# Autodesk Inventor assembly: FRC Fixed Field 2018_sldasm
(part 2 of 4)
- C:\Users\CAD\Documents\GitHub\FIRST-ROBOTICS-2018-5436-CAD\Field\FIRST Power Up Field CAD\Body_858_sldprt.ipt
- C:\Users\CAD\Documents\GitHub\FIRST-ROBOTICS-2018-5436-CAD\Field\FIRST Power Up Field CAD\Body_859_sldprt.ipt
- C:\Users\CAD\Documents\GitHub\FIRST-ROBOTICS-2018-5436-CAD\Field\FIRST Power Up Field CAD\Body_860_sldprt.ipt
- C:\Users\CAD\Documents\GitHub\FIRST-ROBOTICS-2018-5436-CAD\Field\FIRST Power Up Field CAD\Body_861_sldprt.ipt
- C:\Users\CAD\Documents\GitHub\FIRST-ROBOTICS-2018-5436-CAD\Field\FIRST Power Up Field CAD\Body_862_sldprt.ipt
- C:\Users\CAD\Documents\GitHub\FIRST-ROBOTICS-2018-5436-CAD\Field\FIRST Power Up Field CAD\Body_863_sldprt.ipt
- C:\Users\CAD\Documents\GitHub\FIRST-ROBOTICS-2018-5436-CAD\Field\FIRST Power Up Field CAD\Body_864_sldprt.ipt
- C:\Users\CAD\Documents\GitHub\FIRST-ROBOTICS-2018-5436-CAD\Field\FIRST Power Up Field CAD\Body_865_sldprt.ipt
- C:\Users\CAD\Documents\GitHub\FIRST-ROBOTICS-2018-5436-CAD\Field\FIRST Power Up Field CAD\Body_866_sldprt.ipt
- C:\Users\CAD\Documents\GitHub\FIRST-ROBOTICS-2018-5436-CAD\Field\FIRST Power Up Field CAD\Body_867_sldprt.ipt
- C:\Users\CAD\Documents\GitHub\FIRST-ROBOTICS-2018-5436-CAD\Field\FIRST Power Up Field CAD\Body_868_sldprt.ipt
- C:\Users\CAD\Documents\GitHub\FIRST-ROBOTICS-2018-5436-CAD\Field\FIRST Power Up Field CAD\Body_869_sldprt.ipt
- C:\Users\CAD\Documents\GitHub\FIRST-ROBOTICS-2018-5436-CAD\Field\FIRST Power Up Field CAD\Body_870_sldprt.ipt
- C:\Users\CAD\Documents\GitHub\FIRST-ROBOTICS-2018-5436-CAD\Field\FIRST Power Up Field CAD\Body_871_sldprt.ipt
- C:\Users\CAD\Documents\GitHub\FIRST-ROBOTICS-2018-5436-CAD\Field\FIRST Power Up Field CAD\Body_872_sldprt.ipt
- C:\Users\CAD\Documents\GitHub\FIRST-ROBOTICS-2018-5436-CAD\Field\FIRST Power Up Field CAD\Body_873_sldprt.ipt
- C:\Users\CAD\Documents\GitHub\FIRST-ROBOTICS-2018-5436-CAD\Field\FIRST Power Up Field CAD\Body_874_sldprt.ipt
- C:\Users\CAD\Documents\GitHub\FIRST-ROBOTICS-2018-5436-CAD\Field\FIRST Power Up Field CAD\Body_875_sldprt.ipt
- C:\Users\CAD\Documents\GitHub\FIRST-ROBOTICS-2018-5436-CAD\Field\FIRST Power Up Field CAD\Body_876_sldprt.ipt
- C:\Users\CAD\Documents\GitHub\FIRST-ROBOTICS-2018-5436-CAD\Field\FIRST Power Up Field CAD\Body_877_sldprt.ipt
- C:\Users\CAD\Documents\GitHub\FIRST-ROBOTICS-2018-5436-CAD\Field\FIRST Power Up Field CAD\Body_878_sldprt.ipt
- C:\Users\CAD\Documents\GitHub\FIRST-ROBOTICS-2018-5436-CAD\Field\FIRST Power Up Field CAD\Body_879_sldprt.ipt
- C:\Users\CAD\Documents\GitHub\FIRST-ROBOTICS-2018-5436-CAD\Field\FIRST Power Up Field CAD\Body_880_sldprt.ipt
- C:\Users\CAD\Documents\GitHub\FIRST-ROBOTICS-2018-5436-CAD\Field\FIRST Power Up Field CAD\Body_881_sldprt.ipt
- C:\Users\CAD\Documents\GitHub\FIRST-ROBOTICS-2018-5436-CAD\Field\FIRST Power Up Field CAD\Body_882_sldprt.ipt
- C:\Users\CAD\Documents\GitHub\FIRST-ROBOTICS-2018-5436-CAD\Field\FIRST Power Up Field CAD\Body_883_sldprt.ipt
- C:\Users\CAD\Documents\GitHub\FIRST-ROBOTICS-2018-5436-CAD\Field\FIRST Power Up Field CAD\Body_884_sldprt.ipt
- C:\Users\CAD\Documents\GitHub\FIRST-ROBOTICS-2018-5436-CAD\Field\FIRST Power Up Field CAD\Body_885_sldprt.ipt
- C:\Users\CAD\Documents\GitHub\FIRST-ROBOTICS-2018-5436-CAD\Field\FIRST Power Up Field CAD\Body_886_sldprt.ipt
- C:\Users\CAD\Documents\GitHub\FIRST-ROBOTICS-2018-5436-CAD\Field\FIRST Power Up Field CAD\Body_887_sldprt.ipt
- C:\Users\CAD\Documents\GitHub\FIRST-ROBOTICS-2018-5436-CAD\Field\FIRST Power Up Field CAD\Body_888_sldprt.ipt
- C:\Users\CAD\Documents\GitHub\FIRST-ROBOTICS-2018-5436-CAD\Field\FIRST Power Up Field CAD\Body_889_sldprt.ipt
- C:\Users\CAD\Documents\GitHub\FIRST-ROBOTICS-2018-5436-CAD\Field\FIRST Power Up Field CAD\Body_890_sldprt.ipt
- C:\Users\CAD\Documents\GitHub\FIRST-ROBOTICS-2018-5436-CAD\Field\FIRST Power Up Field CAD\Body_891_sldprt.ipt
- C:\Users\CAD\Documents\GitHub\FIRST-ROBOTICS-2018-5436-CAD\Field\FIRST Power Up Field CAD\Body_892_sldprt.ipt
- C:\Users\CAD\Documents\GitHub\FIRST-ROBOTICS-2018-5436-CAD\Field\FIRST Power Up Field CAD\Body_893_sldprt.ipt
- C:\Users\CAD\Documents\GitHub\FIRST-ROBOTICS-2018-5436-CAD\Field\FIRST Power Up Field CAD\Body_894_sldprt.ipt
- C:\Users\CAD\Documents\GitHub\FIRST-ROBOTICS-2018-5436-CAD\Field\FIRST Power Up Field CAD\Body_895_sldprt.ipt
- C:\Users\CAD\Documents\GitHub\FIRST-ROBOTICS-2018-5436-CAD\Field\FIRST Power Up Field CAD\Body_896_sldprt.ipt
- C:\Users\CAD\Documents\GitHub\FIRST-ROBOTICS-2018-5436-CAD\Field\FIRST Power Up Field CAD\Body_897_sldprt.ipt
- C:\Users\CAD\Documents\GitHub\FIRST-ROBOTICS-2018-5436-CAD\Field\FIRST Power Up Field CAD\Body_898_sldprt.ipt
- C:\Users\CAD\Documents\GitHub\FIRST-ROBOTICS-2018-5436-CAD\Field\FIRST Power Up Field CAD\Body_899_sldprt.ipt
- C:\Users\CAD\Documents\GitHub\FIRST-ROBOTICS-2018-5436-CAD\Field\FIRST Power Up Field CAD\Body_900_sldprt.ipt
- C:\Users\CAD\Documents\GitHub\FIRST-ROBOTICS-2018-5436-CAD\Field\FIRST Power Up Field CAD\Body_901_sldprt.ipt
- C:\Users\CAD\Documents\GitHub\FIRST-ROBOTICS-2018-5436-CAD\Field\FIRST Power Up Field CAD\Body_902_sldprt.ipt
- C:\Users\CAD\Documents\GitHub\FIRST-ROBOTICS-2018-5436-CAD\Field\FIRST Power Up Field CAD\Body_903_sldprt.ipt
- C:\Users\CAD\Documents\GitHub\FIRST-ROBOTICS-2018-5436-CAD\Field\FIRST Power Up Field CAD\Body_904_sldprt.ipt
- C:\Users\CAD\Documents\GitHub\FIRST-ROBOTICS-2018-5436-CAD\Field\FIRST Power Up Field CAD\Body_905_sldprt.ipt
- C:\Users\CAD\Documents\GitHub\FIRST-ROBOTICS-2018-5436-CAD\Field\FIRST Power Up Field CAD\Body_906_sldprt.ipt
- C:\Users\CAD\Documents\GitHub\FIRST-ROBOTICS-2018-5436-CAD\Field\FIRST Power Up Field CAD\Body_907_sldprt.ipt
- C:\Users\CAD\Documents\GitHub\FIRST-ROBOTICS-2018-5436-CAD\Field\FIRST Power Up Field CAD\Body_908_sldprt.ipt
- C:\Users\CAD\Documents\GitHub\FIRST-ROBOTICS-2018-5436-CAD\Field\FIRST Power Up Field CAD\Body_909_sldprt.ipt
- C:\Users\CAD\Documents\GitHub\FIRST-ROBOTICS-2018-5436-CAD\Field\FIRST Power Up Field CAD\Body_910_sldprt.ipt
- C:\Users\CAD\Documents\GitHub\FIRST-ROBOTICS-2018-5436-CAD\Field\FIRST Power Up Field CAD\Body_911_sldprt.ipt
- C:\Users\CAD\Documents\GitHub\FIRST-ROBOTICS-2018-5436-CAD\Field\FIRST Power Up Field CAD\Body_912_sldprt.ipt
- C:\Users\CAD\Documents\GitHub\FIRST-ROBOTICS-2018-5436-CAD\Field\FIRST Power Up Field CAD\Body_913_sldprt.ipt
- C:\Users\CAD\Documents\GitHub\FIRST-ROBOTICS-2018-5436-CAD\Field\FIRST Power Up Field CAD\Body_914_sldprt.ipt
- C:\Users\CAD\Documents\GitHub\FIRST-ROBOTICS-2018-5436-CAD\Field\FIRST Power Up Field CAD\Body_915_sldprt.ipt
- C:\Users\CAD\Documents\GitHub\FIRST-ROBOTICS-2018-5436-CAD\Field\FIRST Power Up Field CAD\Body_916_sldprt.ipt
- C:\Users\CAD\Documents\GitHub\FIRST-ROBOTICS-2018-5436-CAD\Field\FIRST Power Up Field CAD\Body_917_sldprt.ipt
- C:\Users\CAD\Documents\GitHub\FIRST-ROBOTICS-2018-5436-CAD\Field\FIRST Power Up Field CAD\Body_918_sldprt.ipt
- C:\Users\CAD\Documents\GitHub\FIRST-ROBOTICS-2018-5436-CAD\Field\FIRST Power Up Field CAD\Body_919_sldprt.ipt
- C:\Users\CAD\Documents\GitHub\FIRST-ROBOTICS-2018-5436-CAD\Field\FIRST Power Up Field CAD\Body_920_sldprt.ipt
- C:\Users\CAD\Documents\GitHub\FIRST-ROBOTICS-2018-5436-CAD\Field\FIRST Power Up Field CAD\Body_921_sldprt.ipt
- C:\Users\CAD\Documents\GitHub\FIRST-ROBOTICS-2018-5436-CAD\Field\FIRST Power Up Field CAD\Body_922_sldprt.ipt
- C:\Users\CAD\Documents\GitHub\FIRST-ROBOTICS-2018-5436-CAD\Field\FIRST Power Up Field CAD\Body_923_sldprt.ipt
- C:\Users\CAD\Documents\GitHub\FIRST-ROBOTICS-2018-5436-CAD\Field\FIRST Power Up Field CAD\Body_924_sldprt.ipt
- C:\Users\CAD\Documents\GitHub\FIRST-ROBOTICS-2018-5436-CAD\Field\FIRST Power Up Field CAD\Body_925_sldprt.ipt
- C:\Users\CAD\Documents\GitHub\FIRST-ROBOTICS-2018-5436-CAD\Field\FIRST Power Up Field CAD\Body_926_sldprt.ipt
- C:\Users\CAD\Documents\GitHub\FIRST-ROBOTICS-2018-5436-CAD\Field\FIRST Power Up Field CAD\Body_927_sldprt.ipt
- C:\Users\CAD\Documents\GitHub\FIRST-ROBOTICS-2018-5436-CAD\Field\FIRST Power Up Field CAD\Body_928_sldprt.ipt
- C:\Users\CAD\Documents\GitHub\FIRST-ROBOTICS-2018-5436-CAD\Field\FIRST Power Up Field CAD\Body_929_sldprt.ipt
- C:\Users\CAD\Documents\GitHub\FIRST-ROBOTICS-2018-5436-CAD\Field\FIRST Power Up Field CAD\Body_930_sldprt.ipt
- C:\Users\CAD\Documents\GitHub\FIRST-ROBOTICS-2018-5436-CAD\Field\FIRST Power Up Field CAD\Body_931_sldprt.ipt
- C:\Users\CAD\Documents\GitHub\FIRST-ROBOTICS-2018-5436-CAD\Field\FIRST Power Up Field CAD\Body_932_sldprt.ipt
- C:\Users\CAD\Documents\GitHub\FIRST-ROBOTICS-2018-5436-CAD\Field\FIRST Power Up Field CAD\Body_933_sldprt.ipt
- C:\Users\CAD\Documents\GitHub\FIRST-ROBOTICS-2018-5436-CAD\Field\FIRST Power Up Field CAD\Body_934_sldprt.ipt
- C:\Users\CAD\Documents\GitHub\FIRST-ROBOTICS-2018-5436-CAD\Field\FIRST Power Up Field CAD\Body_935_sldprt.ipt
- C:\Users\CAD\Documents\GitHub\FIRST-ROBOTICS-2018-5436-CAD\Field\FIRST Power Up Field CAD\Body_936_sldprt.ipt
- C:\Users\CAD\Documents\GitHub\FIRST-ROBOTICS-2018-5436-CAD\Field\FIRST Power Up Field CAD\Body_937_sldprt.ipt
- C:\Users\CAD\Documents\GitHub\FIRST-ROBOTICS-2018-5436-CAD\Field\FIRST Power Up Field CAD\Body_938_sldprt.ipt
- C:\Users\CAD\Documents\GitHub\FIRST-ROBOTICS-2018-5436-CAD\Field\FIRST Power Up Field CAD\Body_939_sldprt.ipt
- C:\Users\CAD\Documents\GitHub\FIRST-ROBOTICS-2018-5436-CAD\Field\FIRST Power Up Field CAD\Body_940_sldprt.ipt
- C:\Users\CAD\Documents\GitHub\FIRST-ROBOTICS-2018-5436-CAD\Field\FIRST Power Up Field CAD\Body_941_sldprt.ipt
- C:\Users\CAD\Documents\GitHub\FIRST-ROBOTICS-2018-5436-CAD\Field\FIRST Power Up Field CAD\Body_942_sldprt.ipt
- C:\Users\CAD\Documents\GitHub\FIRST-ROBOTICS-2018-5436-CAD\Field\FIRST Power Up Field CAD\Body_943_sldprt.ipt
- C:\Users\CAD\Documents\GitHub\FIRST-ROBOTICS-2018-5436-CAD\Field\FIRST Power Up Field CAD\Body_944_sldprt.ipt
- C:\Users\CAD\Documents\GitHub\FIRST-ROBOTICS-2018-5436-CAD\Field\FIRST Power Up Field CAD\Body_945_sldprt.ipt
- C:\Users\CAD\Documents\GitHub\FIRST-ROBOTICS-2018-5436-CAD\Field\FIRST Power Up Field CAD\Body_946_sldprt.ipt
- C:\Users\CAD\Documents\GitHub\FIRST-ROBOTICS-2018-5436-CAD\Field\FIRST Power Up Field CAD\Body_947_sldprt.ipt
- C:\Users\CAD\Documents\GitHub\FIRST-ROBOTICS-2018-5436-CAD\Field\FIRST Power Up Field CAD\Body_948_sldprt.ipt
- C:\Users\CAD\Documents\GitHub\FIRST-ROBOTICS-2018-5436-CAD\Field\FIRST Power Up Field CAD\Body_949_sldprt.ipt
- C:\Users\CAD\Documents\GitHub\FIRST-ROBOTICS-2018-5436-CAD\Field\FIRST Power Up Field CAD\Body_950_sldprt.ipt
- C:\Users\CAD\Documents\GitHub\FIRST-ROBOTICS-2018-5436-CAD\Field\FIRST Power Up Field CAD\Body_951_sldprt.ipt
- C:\Users\CAD\Documents\GitHub\FIRST-ROBOTICS-2018-5436-CAD\Field\FIRST Power Up Field CAD\Body_952_sldprt.ipt
- C:\Users\CAD\Documents\GitHub\FIRST-ROBOTICS-2018-5436-CAD\Field\FIRST Power Up Field CAD\Body_953_sldprt.ipt
- C:\Users\CAD\Documents\GitHub\FIRST-ROBOTICS-2018-5436-CAD\Field\FIRST Power Up Field CAD\Body_954_sldprt.ipt
- C:\Users\CAD\Documents\GitHub\FIRST-ROBOTICS-2018-5436-CAD\Field\FIRST Power Up Field CAD\Body_955_sldprt.ipt
- C:\Users\CAD\Documents\GitHub\FIRST-ROBOTICS-2018-5436-CAD\Field\FIRST Power Up Field CAD\Body_956_sldprt.ipt
- C:\Users\CAD\Documents\GitHub\FIRST-ROBOTICS-2018-5436-CAD\Field\FIRST Power Up Field CAD\Body_957_sldprt.ipt
- C:\Users\CAD\Documents\GitHub\FIRST-ROBOTICS-2018-5436-CAD\Field\FIRST Power Up Field CAD\Body_958_sldprt.ipt
- C:\Users\CAD\Documents\GitHub\FIRST-ROBOTICS-2018-5436-CAD\Field\FIRST Power Up Field CAD\Body_959_sldprt.ipt
- C:\Users\CAD\Documents\GitHub\FIRST-ROBOTICS-2018-5436-CAD\Field\FIRST Power Up Field CAD\Body_960_sldprt.ipt
- C:\Users\CAD\Documents\GitHub\FIRST-ROBOTICS-2018-5436-CAD\Field\FIRST Power Up Field CAD\Body_961_sldprt.ipt
- C:\Users\CAD\Documents\GitHub\FIRST-ROBOTICS-2018-5436-CAD\Field\FIRST Power Up Field CAD\Body_962_sldprt.ipt
- C:\Users\CAD\Documents\GitHub\FIRST-ROBOTICS-2018-5436-CAD\Field\FIRST Power Up Field CAD\Body_963_sldprt.ipt
- C:\Users\CAD\Documents\GitHub\FIRST-ROBOTICS-2018-5436-CAD\Field\FIRST Power Up Field CAD\Body_964_sldprt.ipt
- C:\Users\CAD\Documents\GitHub\FIRST-ROBOTICS-2018-5436-CAD\Field\FIRST Power Up Field CAD\Body_965_sldprt.ipt
- C:\Users\CAD\Documents\GitHub\FIRST-ROBOTICS-2018-5436-CAD\Field\FIRST Power Up Field CAD\Body_966_sldprt.ipt
- C:\Users\CAD\Documents\GitHub\FIRST-ROBOTICS-2018-5436-CAD\Field\FIRST Power Up Field CAD\Body_967_sldprt.ipt
- C:\Users\CAD\Documents\GitHub\FIRST-ROBOTICS-2018-5436-CAD\Field\FIRST Power Up Field CAD\Body_968_sldprt.ipt
- C:\Users\CAD\Documents\GitHub\FIRST-ROBOTICS-2018-5436-CAD\Field\FIRST Power Up Field CAD\Body_969_sldprt.ipt
- C:\Users\CAD\Documents\GitHub\FIRST-ROBOTICS-2018-5436-CAD\Field\FIRST Power Up Field CAD\Body_970_sldprt.ipt
- C:\Users\CAD\Documents\GitHub\FIRST-ROBOTICS-2018-5436-CAD\Field\FIRST Power Up Field CAD\Body_971_sldprt.ipt
- C:\Users\CAD\Documents\GitHub\FIRST-ROBOTICS-2018-5436-CAD\Field\FIRST Power Up Field CAD\Body_972_sldprt.ipt
- C:\Users\CAD\Documents\GitHub\FIRST-ROBOTICS-2018-5436-CAD\Field\FIRST Power Up Field CAD\Body_973_sldprt.ipt
- C:\Users\CAD\Documents\GitHub\FIRST-ROBOTICS-2018-5436-CAD\Field\FIRST Power Up Field CAD\Body_974_sldprt.ipt
- C:\Users\CAD\Documents\GitHub\FIRST-ROBOTICS-2018-5436-CAD\Field\FIRST Power Up Field CAD\Body_975_sldprt.ipt
- C:\Users\CAD\Documents\GitHub\FIRST-ROBOTICS-2018-5436-CAD\Field\FIRST Power Up Field CAD\Body_976_sldprt.ipt
- C:\Users\CAD\Documents\GitHub\FIRST-ROBOTICS-2018-5436-CAD\Field\FIRST Power Up Field CAD\Body_977_sldprt.ipt
- C:\Users\CAD\Documents\GitHub\FIRST-ROBOTICS-2018-5436-CAD\Field\FIRST Power Up Field CAD\Body_978_sldprt.ipt
- C:\Users\CAD\Documents\GitHub\FIRST-ROBOTICS-2018-5436-CAD\Field\FIRST Power Up Field CAD\Body_979_sldprt.ipt
- C:\Users\CAD\Documents\GitHub\FIRST-ROBOTICS-2018-5436-CAD\Field\FIRST Power Up Field CAD\Body_980_sldprt.ipt
- C:\Users\CAD\Documents\GitHub\FIRST-ROBOTICS-2018-5436-CAD\Field\FIRST Power Up Field CAD\Body_981_sldprt.ipt
- C:\Users\CAD\Documents\GitHub\FIRST-ROBOTICS-2018-5436-CAD\Field\FIRST Power Up Field CAD\Body_982_sldprt.ipt
- C:\Users\CAD\Documents\GitHub\FIRST-ROBOTICS-2018-5436-CAD\Field\FIRST Power Up Field CAD\Body_983_sldprt.ipt
- C:\Users\CAD\Documents\GitHub\FIRST-ROBOTICS-2018-5436-CAD\Field\FIRST Power Up Field CAD\Body_984_sldprt.ipt
- C:\Users\CAD\Documents\GitHub\FIRST-ROBOTICS-2018-5436-CAD\Field\FIRST Power Up Field CAD\Body_985_sldprt.ipt
- C:\Users\CAD\Documents\GitHub\FIRST-ROBOTICS-2018-5436-CAD\Field\FIRST Power Up Field CAD\Body_986_sldprt.ipt
- C:\Users\CAD\Documents\GitHub\FIRST-ROBOTICS-2018-5436-CAD\Field\FIRST Power Up Field CAD\Body_987_sldprt.ipt
- C:\Users\CAD\Documents\GitHub\FIRST-ROBOTICS-2018-5436-CAD\Field\FIRST Power Up Field CAD\Body_988_sldprt.ipt
- C:\Users\CAD\Documents\GitHub\FIRST-ROBOTICS-2018-5436-CAD\Field\FIRST Power Up Field CAD\Body_989_sldprt.ipt
- C:\Users\CAD\Documents\GitHub\FIRST-ROBOTICS-2018-5436-CAD\Field\FIRST Power Up Field CAD\Body_990_sldprt.ipt
- C:\Users\CAD\Documents\GitHub\FIRST-ROBOTICS-2018-5436-CAD\Field\FIRST Power Up Field CAD\Body_991_sldprt.ipt
- C:\Users\CAD\Documents\GitHub\FIRST-ROBOTICS-2018-5436-CAD\Field\FIRST Power Up Field CAD\Body_992_sldprt.ipt
- C:\Users\CAD\Documents\GitHub\FIRST-ROBOTICS-2018-5436-CAD\Field\FIRST Power Up Field CAD\Body_993_sldprt.ipt
- C:\Users\CAD\Documents\GitHub\FIRST-ROBOTICS-2018-5436-CAD\Field\FIRST Power Up Field CAD\Body_994_sldprt.ipt
- C:\Users\CAD\Documents\GitHub\FIRST-ROBOTICS-2018-5436-CAD\Field\FIRST Power Up Field CAD\Body_995_sldprt.ipt
- C:\Users\CAD\Documents\GitHub\FIRST-ROBOTICS-2018-5436-CAD\Field\FIRST Power Up Field CAD\Body_996_sldprt.ipt
- C:\Users\CAD\Documents\GitHub\FIRST-ROBOTICS-2018-5436-CAD\Field\FIRST Power Up Field CAD\Body_997_sldprt.ipt
- C:\Users\CAD\Documents\GitHub\FIRST-ROBOTICS-2018-5436-CAD\Field\FIRST Power Up Field CAD\Body_998_sldprt.ipt
- C:\Users\CAD\Documents\GitHub\FIRST-ROBOTICS-2018-5436-CAD\Field\FIRST Power Up Field CAD\Body_999_sldprt.ipt
- C:\Users\CAD\Documents\GitHub\FIRST-ROBOTICS-2018-5436-CAD\Field\FIRST Power Up Field CAD\Body_1000_sldprt.ipt
- C:\Users\CAD\Documents\GitHub\FIRST-ROBOTICS-2018-5436-CAD\Field\FIRST Power Up Field CAD\Body_1001_sldprt.ipt
- C:\Users\CAD\Documents\GitHub\FIRST-ROBOTICS-2018-5436-CAD\Field\FIRST Power Up Field CAD\Body_1002_sldprt.ipt
- C:\Users\CAD\Documents\GitHub\FIRST-ROBOTICS-2018-5436-CAD\Field\FIRST Power Up Field CAD\Body_1003_sldprt.ipt
- C:\Users\CAD\Documents\GitHub\FIRST-ROBOTICS-2018-5436-CAD\Field\FIRST Power Up Field CAD\Body_1004_sldprt.ipt
- C:\Users\CAD\Documents\GitHub\FIRST-ROBOTICS-2018-5436-CAD\Field\FIRST Power Up Field CAD\Body_1005_sldprt.ipt
- C:\Users\CAD\Documents\GitHub\FIRST-ROBOTICS-2018-5436-CAD\Field\FIRST Power Up Field CAD\Body_1006_sldprt.ipt
- C:\Users\CAD\Documents\GitHub\FIRST-ROBOTICS-2018-5436-CAD\Field\FIRST Power Up Field CAD\Body_1007_sldprt.ipt
- C:\Users\CAD\Documents\GitHub\FIRST-ROBOTICS-2018-5436-CAD\Field\FIRST Power Up Field CAD\Body_1008_sldprt.ipt
- C:\Users\CAD\Documents\GitHub\FIRST-ROBOTICS-2018-5436-CAD\Field\FIRST Power Up Field CAD\Body_1009_sldprt.ipt
- C:\Users\CAD\Documents\GitHub\FIRST-ROBOTICS-2018-5436-CAD\Field\FIRST Power Up Field CAD\Body_1010_sldprt.ipt
- C:\Users\CAD\Documents\GitHub\FIRST-ROBOTICS-2018-5436-CAD\Field\FIRST Power Up Field CAD\Body_1011_sldprt.ipt
- C:\Users\CAD\Documents\GitHub\FIRST-ROBOTICS-2018-5436-CAD\Field\FIRST Power Up Field CAD\Body_1012_sldprt.ipt
- C:\Users\CAD\Documents\GitHub\FIRST-ROBOTICS-2018-5436-CAD\Field\FIRST Power Up Field CAD\Body_1013_sldprt.ipt
- C:\Users\CAD\Documents\GitHub\FIRST-ROBOTICS-2018-5436-CAD\Field\FIRST Power Up Field CAD\Body_1014_sldprt.ipt
- C:\Users\CAD\Documents\GitHub\FIRST-ROBOTICS-2018-5436-CAD\Field\FIRST Power Up Field CAD\Body_1015_sldprt.ipt
- C:\Users\CAD\Documents\GitHub\FIRST-ROBOTICS-2018-5436-CAD\Field\FIRST Power Up Field CAD\Body_1016_sldprt.ipt
- C:\Users\CAD\Documents\GitHub\FIRST-ROBOTICS-2018-5436-CAD\Field\FIRST Power Up Field CAD\Body_1017_sldprt.ipt
- C:\Users\CAD\Documents\GitHub\FIRST-ROBOTICS-2018-5436-CAD\Field\FIRST Power Up Field CAD\Body_1018_sldprt.ipt
- C:\Users\CAD\Documents\GitHub\FIRST-ROBOTICS-2018-5436-CAD\Field\FIRST Power Up Field CAD\Body_1019_sldprt.ipt
- C:\Users\CAD\Documents\GitHub\FIRST-ROBOTICS-2018-5436-CAD\Field\FIRST Power Up Field CAD\Body_1020_sldprt.ipt
- C:\Users\CAD\Documents\GitHub\FIRST-ROBOTICS-2018-5436-CAD\Field\FIRST Power Up Field CAD\Body_1021_sldprt.ipt
- C:\Users\CAD\Documents\GitHub\FIRST-ROBOTICS-2018-5436-CAD\Field\FIRST Power Up Field CAD\Body_1022_sldprt.ipt
- C:\Users\CAD\Documents\GitHub\FIRST-ROBOTICS-2018-5436-CAD\Field\FIRST Power Up Field CAD\Body_1023_sldprt.ipt
- C:\Users\CAD\Documents\GitHub\FIRST-ROBOTICS-2018-5436-CAD\Field\FIRST Power Up Field CAD\Body_1024_sldprt.ipt
- C:\Users\CAD\Documents\GitHub\FIRST-ROBOTICS-2018-5436-CAD\Field\FIRST Power Up Field CAD\Body_1025_sldprt.ipt
- C:\Users\CAD\Documents\GitHub\FIRST-ROBOTICS-2018-5436-CAD\Field\FIRST Power Up Field CAD\Body_1026_sldprt.ipt
- C:\Users\CAD\Documents\GitHub\FIRST-ROBOTICS-2018-5436-CAD\Field\FIRST Power Up Field CAD\Body_1027_sldprt.ipt
- C:\Users\CAD\Documents\GitHub\FIRST-ROBOTICS-2018-5436-CAD\Field\FIRST Power Up Field CAD\Body_1028_sldprt.ipt
- C:\Users\CAD\Documents\GitHub\FIRST-ROBOTICS-2018-5436-CAD\Field\FIRST Power Up Field CAD\Body_1029_sldprt.ipt
- C:\Users\CAD\Documents\GitHub\FIRST-ROBOTICS-2018-5436-CAD\Field\FIRST Power Up Field CAD\Body_1030_sldprt.ipt
- C:\Users\CAD\Documents\GitHub\FIRST-ROBOTICS-2018-5436-CAD\Field\FIRST Power Up Field CAD\Body_1031_sldprt.ipt
- C:\Users\CAD\Documents\GitHub\FIRST-ROBOTICS-2018-5436-CAD\Field\FIRST Power Up Field CAD\Body_1032_sldprt.ipt
- C:\Users\CAD\Documents\GitHub\FIRST-ROBOTICS-2018-5436-CAD\Field\FIRST Power Up Field CAD\Body_1033_sldprt.ipt
- C:\Users\CAD\Documents\GitHub\FIRST-ROBOTICS-2018-5436-CAD\Field\FIRST Power Up Field CAD\Body_1034_sldprt.ipt
- C:\Users\CAD\Documents\GitHub\FIRST-ROBOTICS-2018-5436-CAD\Field\FIRST Power Up Field CAD\Body_1035_sldprt.ipt
- C:\Users\CAD\Documents\GitHub\FIRST-ROBOTICS-2018-5436-CAD\Field\FIRST Power Up Field CAD\Body_1036_sldprt.ipt
- C:\Users\CAD\Documents\GitHub\FIRST-ROBOTICS-2018-5436-CAD\Field\FIRST Power Up Field CAD\Body_1037_sldprt.ipt
- C:\Users\CAD\Documents\GitHub\FIRST-ROBOTICS-2018-5436-CAD\Field\FIRST Power Up Field CAD\Body_1038_sldprt.ipt
- C:\Users\CAD\Documents\GitHub\FIRST-ROBOTICS-2018-5436-CAD\Field\FIRST Power Up Field CAD\Body_1039_sldprt.ipt
- C:\Users\CAD\Documents\GitHub\FIRST-ROBOTICS-2018-5436-CAD\Field\FIRST Power Up Field CAD\Body_1040_sldprt.ipt
- C:\Users\CAD\Documents\GitHub\FIRST-ROBOTICS-2018-5436-CAD\Field\FIRST Power Up Field CAD\Body_1041_sldprt.ipt
- C:\Users\CAD\Documents\GitHub\FIRST-ROBOTICS-2018-5436-CAD\Field\FIRST Power Up Field CAD\Body_1042_sldprt.ipt
- C:\Users\CAD\Documents\GitHub\FIRST-ROBOTICS-2018-5436-CAD\Field\FIRST Power Up Field CAD\Body_1043_sldprt.ipt
- C:\Users\CAD\Documents\GitHub\FIRST-ROBOTICS-2018-5436-CAD\Field\FIRST Power Up Field CAD\Body_1044_sldprt.ipt
- C:\Users\CAD\Documents\GitHub\FIRST-ROBOTICS-2018-5436-CAD\Field\FIRST Power Up Field CAD\Body_1045_sldprt.ipt
- C:\Users\CAD\Documents\GitHub\FIRST-ROBOTICS-2018-5436-CAD\Field\FIRST Power Up Field CAD\Body_1046_sldprt.ipt
- C:\Users\CAD\Documents\GitHub\FIRST-ROBOTICS-2018-5436-CAD\Field\FIRST Power Up Field CAD\Body_1047_sldprt.ipt
- C:\Users\CAD\Documents\GitHub\FIRST-ROBOTICS-2018-5436-CAD\Field\FIRST Power Up Field CAD\Body_1048_sldprt.ipt
- C:\Users\CAD\Documents\GitHub\FIRST-ROBOTICS-2018-5436-CAD\Field\FIRST Power Up Field CAD\Body_1049_sldprt.ipt
- C:\Users\CAD\Documents\GitHub\FIRST-ROBOTICS-2018-5436-CAD\Field\FIRST Power Up Field CAD\Body_1050_sldprt.ipt
- C:\Users\CAD\Documents\GitHub\FIRST-ROBOTICS-2018-5436-CAD\Field\FIRST Power Up Field CAD\Body_1051_sldprt.ipt
- C:\Users\CAD\Documents\GitHub\FIRST-ROBOTICS-2018-5436-CAD\Field\FIRST Power Up Field CAD\Body_1052_sldprt.ipt
- C:\Users\CAD\Documents\GitHub\FIRST-ROBOTICS-2018-5436-CAD\Field\FIRST Power Up Field CAD\Body_1053_sldprt.ipt
- C:\Users\CAD\Documents\GitHub\FIRST-ROBOTICS-2018-5436-CAD\Field\FIRST Power Up Field CAD\Body_1054_sldprt.ipt
- C:\Users\CAD\Documents\GitHub\FIRST-ROBOTICS-2018-5436-CAD\Field\FIRST Power Up Field CAD\Body_1055_sldprt.ipt
- C:\Users\CAD\Documents\GitHub\FIRST-ROBOTICS-2018-5436-CAD\Field\FIRST Power Up Field CAD\Body_1056_sldprt.ipt
- C:\Users\CAD\Documents\GitHub\FIRST-ROBOTICS-2018-5436-CAD\Field\FIRST Power Up Field CAD\Body_1057_sldprt.ipt
- C:\Users\CAD\Documents\GitHub\FIRST-ROBOTICS-2018-5436-CAD\Field\FIRST Power Up Field CAD\Body_1058_sldprt.ipt
- C:\Users\CAD\Documents\GitHub\FIRST-ROBOTICS-2018-5436-CAD\Field\FIRST Power Up Field CAD\Body_1059_sldprt.ipt
- C:\Users\CAD\Documents\GitHub\FIRST-ROBOTICS-2018-5436-CAD\Field\FIRST Power Up Field CAD\Body_1060_sldprt.ipt
- C:\Users\CAD\Documents\GitHub\FIRST-ROBOTICS-2018-5436-CAD\Field\FIRST Power Up Field CAD\Body_1061_sldprt.ipt
- C:\Users\CAD\Documents\GitHub\FIRST-ROBOTICS-2018-5436-CAD\Field\FIRST Power Up Field CAD\Body_1062_sldprt.ipt
- C:\Users\CAD\Documents\GitHub\FIRST-ROBOTICS-2018-5436-CAD\Field\FIRST Power Up Field CAD\Body_1063_sldprt.ipt
- C:\Users\CAD\Documents\GitHub\FIRST-ROBOTICS-2018-5436-CAD\Field\FIRST Power Up Field CAD\Body_1064_sldprt.ipt
- C:\Users\CAD\Documents\GitHub\FIRST-ROBOTICS-2018-5436-CAD\Field\FIRST Power Up Field CAD\Body_1065_sldprt.ipt
- C:\Users\CAD\Documents\GitHub\FIRST-ROBOTICS-2018-5436-CAD\Field\FIRST Power Up Field CAD\Body_1066_sldprt.ipt
- C:\Users\CAD\Documents\GitHub\FIRST-ROBOTICS-2018-5436-CAD\Field\FIRST Power Up Field CAD\Body_1067_sldprt.ipt
- C:\Users\CAD\Documents\GitHub\FIRST-ROBOTICS-2018-5436-CAD\Field\FIRST Power Up Field CAD\Body_1068_sldprt.ipt
- C:\Users\CAD\Documents\GitHub\FIRST-ROBOTICS-2018-5436-CAD\Field\FIRST Power Up Field CAD\Body_1069_sldprt.ipt
- C:\Users\CAD\Documents\GitHub\FIRST-ROBOTICS-2018-5436-CAD\Field\FIRST Power Up Field CAD\Body_1070_sldprt.ipt
- C:\Users\CAD\Documents\GitHub\FIRST-ROBOTICS-2018-5436-CAD\Field\FIRST Power Up Field CAD\Body_1071_sldprt.ipt
- C:\Users\CAD\Documents\GitHub\FIRST-ROBOTICS-2018-5436-CAD\Field\FIRST Power Up Field CAD\Body_1072_sldprt.ipt
- C:\Users\CAD\Documents\GitHub\FIRST-ROBOTICS-2018-5436-CAD\Field\FIRST Power Up Field CAD\Body_1073_sldprt.ipt
- C:\Users\CAD\Documents\GitHub\FIRST-ROBOTICS-2018-5436-CAD\Field\FIRST Power Up Field CAD\Body_1074_sldprt.ipt
- C:\Users\CAD\Documents\GitHub\FIRST-ROBOTICS-2018-5436-CAD\Field\FIRST Power Up Field CAD\Body_1075_sldprt.ipt
- C:\Users\CAD\Documents\GitHub\FIRST-ROBOTICS-2018-5436-CAD\Field\FIRST Power Up Field CAD\Body_1076_sldprt.ipt
- C:\Users\CAD\Documents\GitHub\FIRST-ROBOTICS-2018-5436-CAD\Field\FIRST Power Up Field CAD\Body_1077_sldprt.ipt
- C:\Users\CAD\Documents\GitHub\FIRST-ROBOTICS-2018-5436-CAD\Field\FIRST Power Up Field CAD\Body_1078_sldprt.ipt
- C:\Users\CAD\Documents\GitHub\FIRST-ROBOTICS-2018-5436-CAD\Field\FIRST Power Up Field CAD\Body_1079_sldprt.ipt
- C:\Users\CAD\Documents\GitHub\FIRST-ROBOTICS-2018-5436-CAD\Field\FIRST Power Up Field CAD\Body_1080_sldprt.ipt
- C:\Users\CAD\Documents\GitHub\FIRST-ROBOTICS-2018-5436-CAD\Field\FIRST Power Up Field CAD\Body_1081_sldprt.ipt
- C:\Users\CAD\Documents\GitHub\FIRST-ROBOTICS-2018-5436-CAD\Field\FIRST Power Up Field CAD\Body_1082_sldprt.ipt
- C:\Users\CAD\Documents\GitHub\FIRST-ROBOTICS-2018-5436-CAD\Field\FIRST Power Up Field CAD\Body_1083_sldprt.ipt
- C:\Users\CAD\Documents\GitHub\FIRST-ROBOTICS-2018-5436-CAD\Field\FIRST Power Up Field CAD\Body_1084_sldprt.ipt
- C:\Users\CAD\Documents\GitHub\FIRST-ROBOTICS-2018-5436-CAD\Field\FIRST Power Up Field CAD\Body_1085_sldprt.ipt
- C:\Users\CAD\Documents\GitHub\FIRST-ROBOTICS-2018-5436-CAD\Field\FIRST Power Up Field CAD\Body_1086_sldprt.ipt
- C:\Users\CAD\Documents\GitHub\FIRST-ROBOTICS-2018-5436-CAD\Field\FIRST Power Up Field CAD\Body_1087_sldprt.ipt
- C:\Users\CAD\Documents\GitHub\FIRST-ROBOTICS-2018-5436-CAD\Field\FIRST Power Up Field CAD\Body_1088_sldprt.ipt
- C:\Users\CAD\Documents\GitHub\FIRST-ROBOTICS-2018-5436-CAD\Field\FIRST Power Up Field CAD\Body_1089_sldprt.ipt
- C:\Users\CAD\Documents\GitHub\FIRST-ROBOTICS-2018-5436-CAD\Field\FIRST Power Up Field CAD\Body_1090_sldprt.ipt
- C:\Users\CAD\Documents\GitHub\FIRST-ROBOTICS-2018-5436-CAD\Field\FIRST Power Up Field CAD\Body_1091_sldprt.ipt
- C:\Users\CAD\Documents\GitHub\FIRST-ROBOTICS-2018-5436-CAD\Field\FIRST Power Up Field CAD\Body_1092_sldprt.ipt
- C:\Users\CAD\Documents\GitHub\FIRST-ROBOTICS-2018-5436-CAD\Field\FIRST Power Up Field CAD\Body_1093_sldprt.ipt
- C:\Users\CAD\Documents\GitHub\FIRST-ROBOTICS-2018-5436-CAD\Field\FIRST Power Up Field CAD\Body_1094_sldprt.ipt
- C:\Users\CAD\Documents\GitHub\FIRST-ROBOTICS-2018-5436-CAD\Field\FIRST Power Up Field CAD\Body_1095_sldprt.ipt
- C:\Users\CAD\Documents\GitHub\FIRST-ROBOTICS-2018-5436-CAD\Field\FIRST Power Up Field CAD\Body_1096_sldprt.ipt
- C:\Users\CAD\Documents\GitHub\FIRST-ROBOTICS-2018-5436-CAD\Field\FIRST Power Up Field CAD\Body_1097_sldprt.ipt
- C:\Users\CAD\Documents\GitHub\FIRST-ROBOTICS-2018-5436-CAD\Field\FIRST Power Up Field CAD\Body_1098_sldprt.ipt
- C:\Users\CAD\Documents\GitHub\FIRST-ROBOTICS-2018-5436-CAD\Field\FIRST Power Up Field CAD\Body_1099_sldprt.ipt
- C:\Users\CAD\Documents\GitHub\FIRST-ROBOTICS-2018-5436-CAD\Field\FIRST Power Up Field CAD\Body_1100_sldprt.ipt
- C:\Users\CAD\Documents\GitHub\FIRST-ROBOTICS-2018-5436-CAD\Field\FIRST Power Up Field CAD\Body_1101_sldprt.ipt
- C:\Users\CAD\Documents\GitHub\FIRST-ROBOTICS-2018-5436-CAD\Field\FIRST Power Up Field CAD\Body_1102_sldprt.ipt
- C:\Users\CAD\Documents\GitHub\FIRST-ROBOTICS-2018-5436-CAD\Field\FIRST Power Up Field CAD\Body_1103_sldprt.ipt
- C:\Users\CAD\Documents\GitHub\FIRST-ROBOTICS-2018-5436-CAD\Field\FIRST Power Up Field CAD\Body_1104_sldprt.ipt
- C:\Users\CAD\Documents\GitHub\FIRST-ROBOTICS-2018-5436-CAD\Field\FIRST Power Up Field CAD\Body_1105_sldprt.ipt
- C:\Users\CAD\Documents\GitHub\FIRST-ROBOTICS-2018-5436-CAD\Field\FIRST Power Up Field CAD\Body_1106_sldprt.ipt
- C:\Users\CAD\Documents\GitHub\FIRST-ROBOTICS-2018-5436-CAD\Field\FIRST Power Up Field CAD\Body_1107_sldprt.ipt
- C:\Users\CAD\Documents\GitHub\FIRST-ROBOTICS-2018-5436-CAD\Field\FIRST Power Up Field CAD\Body_1108_sldprt.ipt
- C:\Users\CAD\Documents\GitHub\FIRST-ROBOTICS-2018-5436-CAD\Field\FIRST Power Up Field CAD\Body_1109_sldprt.ipt
- C:\Users\CAD\Documents\GitHub\FIRST-ROBOTICS-2018-5436-CAD\Field\FIRST Power Up Field CAD\Body_1110_sldprt.ipt
- C:\Users\CAD\Documents\GitHub\FIRST-ROBOTICS-2018-5436-CAD\Field\FIRST Power Up Field CAD\Body_1111_sldprt.ipt
- C:\Users\CAD\Documents\GitHub\FIRST-ROBOTICS-2018-5436-CAD\Field\FIRST Power Up Field CAD\Body_1112_sldprt.ipt
- C:\Users\CAD\Documents\GitHub\FIRST-ROBOTICS-2018-5436-CAD\Field\FIRST Power Up Field CAD\Body_1113_sldprt.ipt
- C:\Users\CAD\Documents\GitHub\FIRST-ROBOTICS-2018-5436-CAD\Field\FIRST Power Up Field CAD\Body_1114_sldprt.ipt
- C:\Users\CAD\Documents\GitHub\FIRST-ROBOTICS-2018-5436-CAD\Field\FIRST Power Up Field CAD\Body_1115_sldprt.ipt
- C:\Users\CAD\Documents\GitHub\FIRST-ROBOTICS-2018-5436-CAD\Field\FIRST Power Up Field CAD\Body_1116_sldprt.ipt
- C:\Users\CAD\Documents\GitHub\FIRST-ROBOTICS-2018-5436-CAD\Field\FIRST Power Up Field CAD\Body_1117_sldprt.ipt
- C:\Users\CAD\Documents\GitHub\FIRST-ROBOTICS-2018-5436-CAD\Field\FIRST Power Up Field CAD\Body_1118_sldprt.ipt
- C:\Users\CAD\Documents\GitHub\FIRST-ROBOTICS-2018-5436-CAD\Field\FIRST Power Up Field CAD\Body_1119_sldprt.ipt
- C:\Users\CAD\Documents\GitHub\FIRST-ROBOTICS-2018-5436-CAD\Field\FIRST Power Up Field CAD\Body_1120_sldprt.ipt
- C:\Users\CAD\Documents\GitHub\FIRST-ROBOTICS-2018-5436-CAD\Field\FIRST Power Up Field CAD\Body_1121_sldprt.ipt
- C:\Users\CAD\Documents\GitHub\FIRST-ROBOTICS-2018-5436-CAD\Field\FIRST Power Up Field CAD\Body_1122_sldprt.ipt
- C:\Users\CAD\Documents\GitHub\FIRST-ROBOTICS-2018-5436-CAD\Field\FIRST Power Up Field CAD\Body_1123_sldprt.ipt
- C:\Users\CAD\Documents\GitHub\FIRST-ROBOTICS-2018-5436-CAD\Field\FIRST Power Up Field CAD\Body_1124_sldprt.ipt
- C:\Users\CAD\Documents\GitHub\FIRST-ROBOTICS-2018-5436-CAD\Field\FIRST Power Up Field CAD\Body_1125_sldprt.ipt
- C:\Users\CAD\Documents\GitHub\FIRST-ROBOTICS-2018-5436-CAD\Field\FIRST Power Up Field CAD\Body_1126_sldprt.ipt
- C:\Users\CAD\Documents\GitHub\FIRST-ROBOTICS-2018-5436-CAD\Field\FIRST Power Up Field CAD\Body_1127_sldprt.ipt
- C:\Users\CAD\Documents\GitHub\FIRST-ROBOTICS-2018-5436-CAD\Field\FIRST Power Up Field CAD\Body_1128_sldprt.ipt
- C:\Users\CAD\Documents\GitHub\FIRST-ROBOTICS-2018-5436-CAD\Field\FIRST Power Up Field CAD\Body_1129_sldprt.ipt
- C:\Users\CAD\Documents\GitHub\FIRST-ROBOTICS-2018-5436-CAD\Field\FIRST Power Up Field CAD\Body_1130_sldprt.ipt
- C:\Users\CAD\Documents\GitHub\FIRST-ROBOTICS-2018-5436-CAD\Field\FIRST Power Up Field CAD\Body_1131_sldprt.ipt
- C:\Users\CAD\Documents\GitHub\FIRST-ROBOTICS-2018-5436-CAD\Field\FIRST Power Up Field CAD\Body_1132_sldprt.ipt
- C:\Users\CAD\Documents\GitHub\FIRST-ROBOTICS-2018-5436-CAD\Field\FIRST Power Up Field CAD\Body_1133_sldprt.ipt
- C:\Users\CAD\Documents\GitHub\FIRST-ROBOTICS-2018-5436-CAD\Field\FIRST Power Up Field CAD\Body_1134_sldprt.ipt
- C:\Users\CAD\Documents\GitHub\FIRST-ROBOTICS-2018-5436-CAD\Field\FIRST Power Up Field CAD\Body_1135_sldprt.ipt
- C:\Users\CAD\Documents\GitHub\FIRST-ROBOTICS-2018-5436-CAD\Field\FIRST Power Up Field CAD\Body_1136_sldprt.ipt
- C:\Users\CAD\Documents\GitHub\FIRST-ROBOTICS-2018-5436-CAD\Field\FIRST Power Up Field CAD\Body_1137_sldprt.ipt
- C:\Users\CAD\Documents\GitHub\FIRST-ROBOTICS-2018-5436-CAD\Field\FIRST Power Up Field CAD\Body_1138_sldprt.ipt
- C:\Users\CAD\Documents\GitHub\FIRST-ROBOTICS-2018-5436-CAD\Field\FIRST Power Up Field CAD\Body_1139_sldprt.ipt
- C:\Users\CAD\Documents\GitHub\FIRST-ROBOTICS-2018-5436-CAD\Field\FIRST Power Up Field CAD\Body_1140_sldprt.ipt
- C:\Users\CAD\Documents\GitHub\FIRST-ROBOTICS-2018-5436-CAD\Field\FIRST Power Up Field CAD\Body_1141_sldprt.ipt
- C:\Users\CAD\Documents\GitHub\FIRST-ROBOTICS-2018-5436-CAD\Field\FIRST Power Up Field CAD\Body_1142_sldprt.ipt
- C:\Users\CAD\Documents\GitHub\FIRST-ROBOTICS-2018-5436-CAD\Field\FIRST Power Up Field CAD\Body_1143_sldprt.ipt
- C:\Users\CAD\Documents\GitHub\FIRST-ROBOTICS-2018-5436-CAD\Field\FIRST Power Up Field CAD\Body_1144_sldprt.ipt
- C:\Users\CAD\Documents\GitHub\FIRST-ROBOTICS-2018-5436-CAD\Field\FIRST Power Up Field CAD\Body_1145_sldprt.ipt
- C:\Users\CAD\Documents\GitHub\FIRST-ROBOTICS-2018-5436-CAD\Field\FIRST Power Up Field CAD\Body_1146_sldprt.ipt
- C:\Users\CAD\Documents\GitHub\FIRST-ROBOTICS-2018-5436-CAD\Field\FIRST Power Up Field CAD\Body_1147_sldprt.ipt
- C:\Users\CAD\Documents\GitHub\FIRST-ROBOTICS-2018-5436-CAD\Field\FIRST Power Up Field CAD\Body_1148_sldprt.ipt
- C:\Users\CAD\Documents\GitHub\FIRST-ROBOTICS-2018-5436-CAD\Field\FIRST Power Up Field CAD\Body_1149_sldprt.ipt
- C:\Users\CAD\Documents\GitHub\FIRST-ROBOTICS-2018-5436-CAD\Field\FIRST Power Up Field CAD\Body_1150_sldprt.ipt
- C:\Users\CAD\Documents\GitHub\FIRST-ROBOTICS-2018-5436-CAD\Field\FIRST Power Up Field CAD\Body_1151_sldprt.ipt
- C:\Users\CAD\Documents\GitHub\FIRST-ROBOTICS-2018-5436-CAD\Field\FIRST Power Up Field CAD\Body_1152_sldprt.ipt
- C:\Users\CAD\Documents\GitHub\FIRST-ROBOTICS-2018-5436-CAD\Field\FIRST Power Up Field CAD\Body_1153_sldprt.ipt
- C:\Users\CAD\Documents\GitHub\FIRST-ROBOTICS-2018-5436-CAD\Field\FIRST Power Up Field CAD\Body_1154_sldprt.ipt
- C:\Users\CAD\Documents\GitHub\FIRST-ROBOTICS-2018-5436-CAD\Field\FIRST Power Up Field CAD\Body_1155_sldprt.ipt
- C:\Users\CAD\Documents\GitHub\FIRST-ROBOTICS-2018-5436-CAD\Field\FIRST Power Up Field CAD\Body_1156_sldprt.ipt
- C:\Users\CAD\Documents\GitHub\FIRST-ROBOTICS-2018-5436-CAD\Field\FIRST Power Up Field CAD\Body_1157_sldprt.ipt
- C:\Users\CAD\Documents\GitHub\FIRST-ROBOTICS-2018-5436-CAD\Field\FIRST Power Up Field CAD\Body_1158_sldprt.ipt
- C:\Users\CAD\Documents\GitHub\FIRST-ROBOTICS-2018-5436-CAD\Field\FIRST Power Up Field CAD\Body_1159_sldprt.ipt
- C:\Users\CAD\Documents\GitHub\FIRST-ROBOTICS-2018-5436-CAD\Field\FIRST Power Up Field CAD\Body_1160_sldprt.ipt
- C:\Users\CAD\Documents\GitHub\FIRST-ROBOTICS-2018-5436-CAD\Field\FIRST Power Up Field CAD\Body_1161_sldprt.ipt
- C:\Users\CAD\Documents\GitHub\FIRST-ROBOTICS-2018-5436-CAD\Field\FIRST Power Up Field CAD\Body_1162_sldprt.ipt
- C:\Users\CAD\Documents\GitHub\FIRST-ROBOTICS-2018-5436-CAD\Field\FIRST Power Up Field CAD\Body_1163_sldprt.ipt
- C:\Users\CAD\Documents\GitHub\FIRST-ROBOTICS-2018-5436-CAD\Field\FIRST Power Up Field CAD\Body_1164_sldprt.ipt
- C:\Users\CAD\Documents\GitHub\FIRST-ROBOTICS-2018-5436-CAD\Field\FIRST Power Up Field CAD\Body_1165_sldprt.ipt
- C:\Users\CAD\Documents\GitHub\FIRST-ROBOTICS-2018-5436-CAD\Field\FIRST Power Up Field CAD\Body_1166_sldprt.ipt
- C:\Users\CAD\Documents\GitHub\FIRST-ROBOTICS-2018-5436-CAD\Field\FIRST Power Up Field CAD\Body_1167_sldprt.ipt
- C:\Users\CAD\Documents\GitHub\FIRST-ROBOTICS-2018-5436-CAD\Field\FIRST Power Up Field CAD\Body_1168_sldprt.ipt
- C:\Users\CAD\Documents\GitHub\FIRST-ROBOTICS-2018-5436-CAD\Field\FIRST Power Up Field CAD\Body_1169_sldprt.ipt
- C:\Users\CAD\Documents\GitHub\FIRST-ROBOTICS-2018-5436-CAD\Field\FIRST Power Up Field CAD\Body_1170_sldprt.ipt
- C:\Users\CAD\Documents\GitHub\FIRST-ROBOTICS-2018-5436-CAD\Field\FIRST Power Up Field CAD\Body_1171_sldprt.ipt
- C:\Users\CAD\Documents\GitHub\FIRST-ROBOTICS-2018-5436-CAD\Field\FIRST Power Up Field CAD\Body_1172_sldprt.ipt
- C:\Users\CAD\Documents\GitHub\FIRST-ROBOTICS-2018-5436-CAD\Field\FIRST Power Up Field CAD\Body_1173_sldprt.ipt
- C:\Users\CAD\Documents\GitHub\FIRST-ROBOTICS-2018-5436-CAD\Field\FIRST Power Up Field CAD\Body_1174_sldprt.ipt
- C:\Users\CAD\Documents\GitHub\FIRST-ROBOTICS-2018-5436-CAD\Field\FIRST Power Up Field CAD\Body_1175_sldprt.ipt
- C:\Users\CAD\Documents\GitHub\FIRST-ROBOTICS-2018-5436-CAD\Field\FIRST Power Up Field CAD\Body_1176_sldprt.ipt
- C:\Users\CAD\Documents\GitHub\FIRST-ROBOTICS-2018-5436-CAD\Field\FIRST Power Up Field CAD\Body_1177_sldprt.ipt
- C:\Users\CAD\Documents\GitHub\FIRST-ROBOTICS-2018-5436-CAD\Field\FIRST Power Up Field CAD\Body_1178_sldprt.ipt
- C:\Users\CAD\Documents\GitHub\FIRST-ROBOTICS-2018-5436-CAD\Field\FIRST Power Up Field CAD\Body_1179_sldprt.ipt
- C:\Users\CAD\Documents\GitHub\FIRST-ROBOTICS-2018-5436-CAD\Field\FIRST Power Up Field CAD\Body_1180_sldprt.ipt
- C:\Users\CAD\Documents\GitHub\FIRST-ROBOTICS-2018-5436-CAD\Field\FIRST Power Up Field CAD\Body_1181_sldprt.ipt
- C:\Users\CAD\Documents\GitHub\FIRST-ROBOTICS-2018-5436-CAD\Field\FIRST Power Up Field CAD\Body_1182_sldprt.ipt
- C:\Users\CAD\Documents\GitHub\FIRST-ROBOTICS-2018-5436-CAD\Field\FIRST Power Up Field CAD\Body_1183_sldprt.ipt
- C:\Users\CAD\Documents\GitHub\FIRST-ROBOTICS-2018-5436-CAD\Field\FIRST Power Up Field CAD\Body_1184_sldprt.ipt
- C:\Users\CAD\Documents\GitHub\FIRST-ROBOTICS-2018-5436-CAD\Field\FIRST Power Up Field CAD\Body_1185_sldprt.ipt
- C:\Users\CAD\Documents\GitHub\FIRST-ROBOTICS-2018-5436-CAD\Field\FIRST Power Up Field CAD\Body_1186_sldprt.ipt
- C:\Users\CAD\Documents\GitHub\FIRST-ROBOTICS-2018-5436-CAD\Field\FIRST Power Up Field CAD\Body_1187_sldprt.ipt
- C:\Users\CAD\Documents\GitHub\FIRST-ROBOTICS-2018-5436-CAD\Field\FIRST Power Up Field CAD\Body_1188_sldprt.ipt
- C:\Users\CAD\Documents\GitHub\FIRST-ROBOTICS-2018-5436-CAD\Field\FIRST Power Up Field CAD\Body_1189_sldprt.ipt
- C:\Users\CAD\Documents\GitHub\FIRST-ROBOTICS-2018-5436-CAD\Field\FIRST Power Up Field CAD\Body_1190_sldprt.ipt
- C:\Users\CAD\Documents\GitHub\FIRST-ROBOTICS-2018-5436-CAD\Field\FIRST Power Up Field CAD\Body_1191_sldprt.ipt
- C:\Users\CAD\Documents\GitHub\FIRST-ROBOTICS-2018-5436-CAD\Field\FIRST Power Up Field CAD\Body_1192_sldprt.ipt